# Autodesk Inventor assembly: XM430_ASM_WITHOUT-BACK
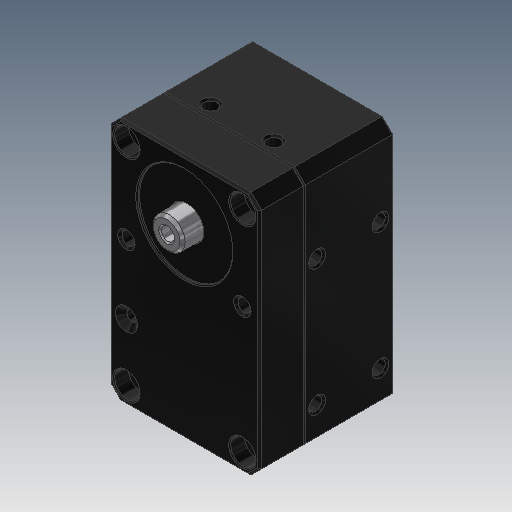
[picture p0: Inventor's stored thumbnail of the model, 512x512]
Saved by Autodesk Inventor 2019.4 (Build 234330000, 330)
## iProperties
Created: 2019-10-08
Part Number: XM430_ASM_WITHOUT-BACK
Material: 一般
Document SubType Name: Assembly
Designer: y6tada
Author: y6tada
## Documents named in this file (3)
- C:\GrabCAD\Yunit 8\Libs\DYNAMIXEL\XM430\XM430_ASM_WITHOUT-BACK.iam
- C:\GrabCAD\Yunit 8\Libs\DYNAMIXEL\XM430\XM430_HOUSING_MIDDLE.ipt
- C:\GrabCAD\Yunit 8\Libs\DYNAMIXEL\XM430\XM430_HOUSING_TOP.ipt
## Components (2 placed, 2 different names)
1. XM430_HOUSING_MIDDLE:1 — フラッシュ:1, フラッシュ:2, フラッシュ:3, フラッシュ:4, フラッシュ:5, メイト:1
2. XM430_HOUSING_TOP:1 — フラッシュ:4, フラッシュ:5, メイト:1
## Relationships (6: Flush 5, Mate 1)
- フラッシュ:1 [Flush]: XM430_HOUSING_MIDDLE:1
- フラッシュ:2 [Flush]: XM430_HOUSING_MIDDLE:1
- フラッシュ:3 [Flush]: XM430_HOUSING_MIDDLE:1
- フラッシュ:4 [Flush]: XM430_HOUSING_MIDDLE:1 ↔ XM430_HOUSING_TOP:1
- フラッシュ:5 [Flush]: XM430_HOUSING_MIDDLE:1 ↔ XM430_HOUSING_TOP:1
- メイト:1 [Mate]: XM430_HOUSING_MIDDLE:1 ↔ XM430_HOUSING_TOP:1
